# Autodesk Inventor assembly: Zespół1
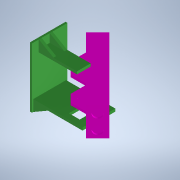
[picture p0: Inventor's stored thumbnail of the model, 180x180]
Saved by Autodesk Inventor 2022.2 (Build 262287010, 287A)
## iProperties
Created: 2023-01-23
Part Number: Zespół1
Document SubType Name: Assembly
Designer: Miki
Author: Miki
## Documents named in this file (3)
- C:\Users\Miki\Desktop\SM_ROWNIA\Zespół1.iam
- C:\Users\Miki\Desktop\SM_ROWNIA\Część1.ipt
- C:\Users\Miki\Desktop\SM_ROWNIA\Część2.ipt
## Components (2 placed, 2 different names)
1. Część1:1 — Zestawiające:1, Walcowe:2
2. Część2:1 — Zestawiające:1, Walcowe:2
## Relationships (2: Mate 1, CylindricalJoint 1)
- Zestawiające:1 [Mate] (1 mm): Część1:1 ↔ Część2:1
- Walcowe:2 [CylindricalJoint]: Część1:1 ↔ Część2:1
